# Autodesk Inventor assembly: Rover
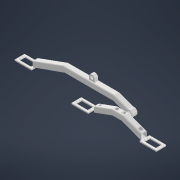
[picture p0: Inventor's stored thumbnail of the model, 180x180]
Saved by Autodesk Inventor 2021 (Build 250183000, 183)
## iProperties
Created: 2021-01-03
Part Number: Rover
Document SubType Name: Assembly
Designer: laure
Author: laure
## Documents named in this file (5)
- E:\Projects\Rover\Rover.iam
- E:\Projects\Rover\Rocker_hinten.ipt
- E:\Projects\Rover\Rocker_vorne.ipt
- E:\Projects\Rover\Bogie.ipt
- E:\Projects\Rover\Servohalterung_v2.ipt
## Components (6 placed, 4 different names)
1. Fahrwerk_rocker_hinten:1 — Passend:2, Passend:3, Winkel:1
2. Fahrwerk_rocker_vorne:1
3. Fahrwerk_bogie:1 — Passend:2, Passend:3, Winkel:1
4. Servohalterung_v2:1
5. Servohalterung_v2:2
6. Servohalterung_v2:3
## Relationships (3: Mate 2, Angle 1)
- Passend:2 [Mate]: Fahrwerk_rocker_hinten:1 ↔ Fahrwerk_bogie:1
- Passend:3 [Mate]: Fahrwerk_rocker_hinten:1 ↔ Fahrwerk_bogie:1
- Winkel:1 [Angle] (0 deg): Fahrwerk_rocker_hinten:1 ↔ Fahrwerk_bogie:1
